# Autodesk Inventor assembly: fc18-037
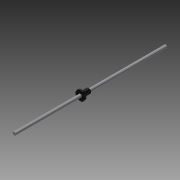
[picture p0: Inventor's stored thumbnail of the model, 180x180]
Saved by Autodesk Inventor 2018 (Build 220112000, 112)
## iProperties
Category: Miscellaneous
Company: Autodesk Inc.
Created: 2017-11-23
Part Number: fc18-037
Document SubType Name: Assembly
Designer: Autodesk Inc.
Catalog Web Link: http://www.haydonkerk.com/LinearActuatorProducts/LeadScrewsAndNuts/LeadScrews/tabid/108/Default.aspx
Vendor: Haydon Kerk Motion Solutions
Author: Autodesk Inc.
Keywords: FIRSTChoice
## Documents named in this file (3)
- F:\FIRST 2018\FIRST 2018 FirstChoice\fc18-037_LeadScrew.iam
- F:\FIRST 2018\FIRST 2018 FirstChoice\Parts\Ametek-BFWFNR-037-1000-18_1.ipt
- F:\FIRST 2018\FIRST 2018 FirstChoice\Parts\Ametek-BFWFNR-037-1000-18_2.ipt
## Components (2 placed, 2 different names)
1. Ametek-BFWFNR-037-1000-18_1:1 — Mate:1
2. Ametek-BFWFNR-037-1000-18_2:1 — Mate:1
## Relationships (1: Mate 1)
- Mate:1: Ametek-BFWFNR-037-1000-18_1:1 ↔ Ametek-BFWFNR-037-1000-18_2:1
